# Autodesk Inventor assembly: teste suporte
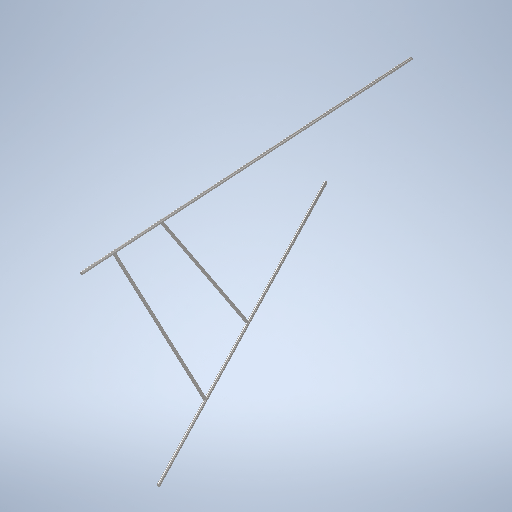
[picture p0: Inventor's stored thumbnail of the model, 512x512]
Saved by Autodesk Inventor 2025.1 (Build 291241000, 241)
## iProperties
Created: 2024-11-05
Part Number: teste suporte
Document SubType Name: Assembly
Designer: pedro
Author: pedro
## Documents named in this file (3)
- C:\Users\pedro\Documents\1-CoisasSerias\UTFPR\2024-2\Oficina\Estrutura\teste suporte.iam
- C:\Users\pedro\Documents\1-CoisasSerias\UTFPR\2024-2\Oficina\Estrutura\Pecas Prontas\impressora-3d-12.snapshot.2\impressora 3.0\Guia Linear 490mm.ipt
- C:\Users\pedro\Documents\1-CoisasSerias\UTFPR\2024-2\Oficina\Estrutura\Pecas Prontas\impressora-3d-12.snapshot.2\impressora 3.0\Guia Linear 480mm.ipt
## Components (4 placed, 2 different names)
1. Guia Linear 965mm:1 — Coincidente:2
2. Guia Linear 965mm:2
3. Guia Linear 480mm:1
4. Guia Linear 480mm:2 — Coincidente:2
## Relationships (1: Mate 1)
- Coincidente:2 [Mate]: Guia Linear 965mm:1 ↔ Guia Linear 480mm:2
